# Autodesk Inventor assembly: Foot_for_rotation
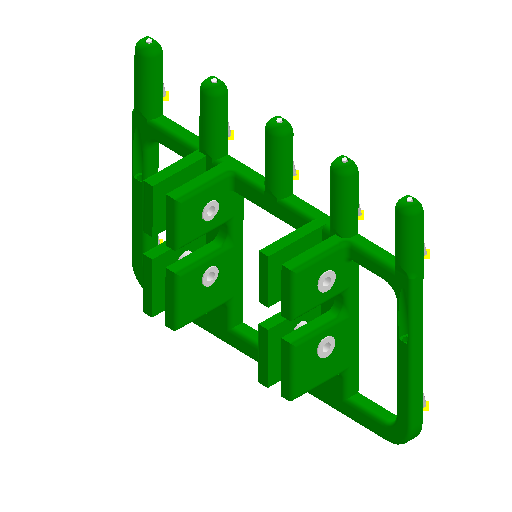
[picture p0: Inventor's stored thumbnail of the model, 512x512]
Saved by Autodesk Inventor 2023.1 (Build 271208000, 208)
## iProperties
Created: 2023-05-17
Part Number: Foot_for_rotation
Document SubType Name: Assembly
Designer: Windows10
Author: Windows10
## Documents named in this file (5)
- C:\Users\Windows10\Dropbox\Study\Climbing_Robot\CAD\new_robot_model\Foot_for_rotation.iam
- C:\Users\Windows10\Dropbox\Study\Climbing_Robot\CAD\new_robot_model\Passivfeet_big_more_Claws_MIR1.ipt
- C:\Users\Windows10\Dropbox\Study\Climbing_Robot\CAD\new_robot_model\Shaft_Rotational_Joints_Feet_MIR2.ipt
- C:\Users\Windows10\Dropbox\Study\Climbing_Robot\CAD\new_robot_model\Shaft_Rotational_Joints_Feet_MIR_MIR1.ipt
- C:\Users\Windows10\Dropbox\Study\Climbing_Robot\CAD\new_robot_model\foot_claw_2.5_MIR1.ipt
## Components (12 placed, 4 different names)
1. Passivfeet_big_more_Claws_MIR1:1
2. Shaft_Rotational_Joints_Feet_MIR2:1
3. Shaft_Rotational_Joints_Feet_MIR2:2
4. Shaft_Rotational_Joints_Feet_MIR_MIR1:1
5. Shaft_Rotational_Joints_Feet_MIR_MIR1:2
6. foot_claw_2.5_MIR1:1
7. foot_claw_2.5_MIR1:2
8. foot_claw_2.5_MIR1:3
9. foot_claw_2.5_MIR1:4
10. foot_claw_2.5_MIR1:5
11. foot_claw_2.5_MIR1:6
12. foot_claw_2.5_MIR1:7
## Relationships (4: Insert 2, Mate 2)
- [Insert] (-9 mm): Passivfeet_big_more_Claws_MIR1:1 ↔ Shaft_Rotational_Joints_Feet_MIR2:1
- [Insert] (-9 mm): Passivfeet_big_more_Claws_MIR1:1 ↔ Shaft_Rotational_Joints_Feet_MIR2:2
- [Mate]: Passivfeet_big_more_Claws_MIR1:1 ↔ Shaft_Rotational_Joints_Feet_MIR_MIR1:2
- [Mate]: Passivfeet_big_more_Claws_MIR1:1 ↔ Shaft_Rotational_Joints_Feet_MIR_MIR1:1
